# Autodesk Inventor assembly: 長穴減速_ホーン_2
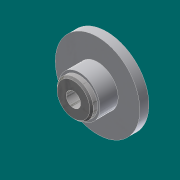
[picture p0: Inventor's stored thumbnail of the model, 180x180]
Saved by Autodesk Inventor 2016 (Build 200138000, 138)
## iProperties
Created: 2016-08-26
Part Number: 長穴減速_ホーン_2
Material: 一般
Document SubType Name: Assembly
Designer: hiro
Author: hiro
## Documents named in this file (3)
- C:\Users\hiro\Documents\kenkyuu\二足\二足ver6.0\下半身_160823\リンク\長穴減速_ホーン_2.iam
- C:\Users\hiro\Documents\kenkyuu\二足\二足ver6.0\既製品\新規購入\D6068-4530.ipt
- C:\Users\hiro\Documents\kenkyuu\二足\二足ver6.0\既製品\新規購入\ARU-305_5.ipt
## Components (2 placed, 2 different names)
1. D6068-4530:1 — 挿入:1, メイト:1, メイト:2, フラッシュ:4
2. ARU-305_5:1 — 挿入:1
## Relationships (4: Mate 2, Insert 1, Flush 1)
- 挿入:1 [Insert]: D6068-4530:1 ↔ ARU-305_5:1
- メイト:1 [Mate]: D6068-4530:1
- メイト:2 [Mate]: D6068-4530:1
- フラッシュ:4 [Flush]: D6068-4530:1
